# Autodesk Inventor assembly: 21308 E
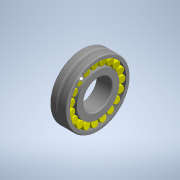
[picture p0: Inventor's stored thumbnail of the model, 180x180]
Saved by Autodesk Inventor 2021 (Build 250183000, 183)
## iProperties
Category: PARTsolutions
Company: SKF
Part Number: 21308 E
Catalog Web Link: www.cadenas.de
Description: BS2_001-Spherical roller bearings
Vendor: SKF
Document SubType Name: Assembly
Designer: partserver
Manufacturer: SKF
Mass: 740 g
Surface Area: 404.704 cm^2
Volume: 89.5824 cm^3
Density: 8.26055 g/cm^3
PSOL_IDENT_0: {$CADENAS_DATA\23d-libs\skf\bearings_units_and_housings\roller_bearings\spherical_roller_bearings\bs
PSOL_IDENT_1: 2_001.prj},173 {VTYP=3D},{STYP=ASSTAB},{NB=21308 E},{LINA=21308 E},{NN=BS2_001},{DATE=23.12.2020 07:
PSOL_IDENT_2: 01:43},{GEOMDATE=14.12.2020 11:44:40},{VERSION=},{LINEID=461840},{WBVAR=},{WBNUMERIC=}  {NB=21308 E}
PSOL_IDENT_3: ,{LINA=21308 E},{KT=DUMMY},{DESIGNATION=21308 E},{VARIANT=CE1W33},{DESIGNX=Cylindrical bore},{SEAL=N
PSOL_IDENT_4: o seals},{SALG=NO},{BORE=40.000},{DD=40.000},{DD1=MIN},{D=90.000},{B=23.000},{DD2=60.000},{DD3=MIN},
PSOL_IDENT_5: {D1=79.800},{B1=MIN},{B2=MIN},{B4=MIN},{B5=MIN},{BB=5.500},{K=3.000},{R12=1.500},{G=},{G1=MIN},{TB=M
PSOL_IDENT_6: IN},{ALPHA=9.0833},{R34=MIN},{PITCH=71.097},{DW=10.200},{LW=8.400},{DDAMIN=49.000},{DDAMAX=MIN},{DBM
PSOL_IDENT_7: IN=MIN},{DAMAX=81.000},{BAMIN=MIN},{RAMAX=1.500},{LOAD1=107.000},{LOAD2=108.000},{LOAD3=11.800},{SPE
PSOL_IDENT_8: ED1=7000},{SPEED2=9500},{PRA=},{PLA=},{Z=19.000},{II=2.000},{MASS=0.740},{MASS2=MIN},{SLEEVE=},{POPU
PSOL_IDENT_9: LAR=Yes},{BEARING=21308 E},{PPATH=parts/bs2_001_asmtpl.prj},{RAMAXX=1.5},{EE=0.24},{Y0=2.8},{R12X=1.
PSOL_IDENT_10: 5},{Y2=4.2},{ALPHAX=9.08333},{Y1=2.8},{DD1X=},{B1X=},{SLEEVEX=},{ALPHAXX=},{B2X=},{SUPRESSED=},{BBAL
PSOL_IDENT_11: G=5.500},{KALG=3.000}
NB: 21308 E
NN: BS2_001
NT: Spherical roller bearings
NBSYN: $DESIGNATION.
LINA: 21308 E
CATALOG: SKF
DESIGNATION: 21308 E
DESIGNX: Cylindrical bore
SEAL: No seals
BORE: 40
D: 90
B: 23
LOAD1: 107
LOAD2: 108
LOAD3: 11.8
SPEED1: 7000
SPEED2: 9500
SUPPLIER: SKF
ARTICLENO: 21308 E
BOMINFO: 21308 E
CREATOR: CADENAS GmbH
Title: 21308 E
Author: Cadenas PARTsolutions
Comments: Spherical roller bearings
## Documents named in this file (6)
- C:\Users\Διογενης Τσιχλακης\Documents\Inventor\GearBoxTurboProp\21308 E.iam
- C:\Users\Διογενης Τσιχλακης\Documents\Inventor\GearBoxTurboProp\21308 E_dummy.ipt
- C:\Users\Διογενης Τσιχλακης\Documents\Inventor\GearBoxTurboProp\21308 E_ir.ipt
- C:\Users\Διογενης Τσιχλακης\Documents\Inventor\GearBoxTurboProp\21308 E_or.ipt
- C:\Users\Διογενης Τσιχλακης\Documents\Inventor\GearBoxTurboProp\21308 E_r1.ipt
- C:\Users\Διογενης Τσιχλακης\Documents\Inventor\GearBoxTurboProp\21308 E_r2.ipt
## Components (41 placed, 5 different names)
1. 21308 E_dummy:1 — dummy_XY@1 <-> ir_XY@2, dummy_Z@1 <-> ir_Z@2, dummy_YZ@1 <-> ir_YZ@2, dummy_YZ@1 <-> or_YZ@3, roller1_XY@1 <-> roller1_XY@4, roller1_Z@1 <-> roller1_Z@4, roller1_YZ@1 <-> roller1_YZ@4, roller1_XY@1 <-> roller2_XY@5, roller1_Z@1 <-> roller2_Z@5, roller1_YZ@1 <-> roller2_YZ@5, roller2_XY@1 <-> roller1_XY@6, roller2_Z@1 <-> roller1_Z@6, roller2_YZ@1 <-> roller1_YZ@6, roller2_XY@1 <-> roller2_XY@7, roller2_Z@1 <-> roller2_Z@7, roller2_YZ@1 <-> roller2_YZ@7, roller3_XY@1 <-> roller1_XY@8, roller3_Z@1 <-> roller1_Z@8, roller3_YZ@1 <-> roller1_YZ@8, roller3_XY@1 <-> roller2_XY@9, roller3_Z@1 <-> roller2_Z@9, roller3_YZ@1 <-> roller2_YZ@9, roller4_XY@1 <-> roller1_XY@10, roller4_Z@1 <-> roller1_Z@10, roller4_YZ@1 <-> roller1_YZ@10, roller4_XY@1 <-> roller2_XY@11, roller4_Z@1 <-> roller2_Z@11, roller4_YZ@1 <-> roller2_YZ@11, roller5_XY@1 <-> roller1_XY@12, roller5_Z@1 <-> roller1_Z@12, roller5_YZ@1 <-> roller1_YZ@12, roller5_XY@1 <-> roller2_XY@13, roller5_Z@1 <-> roller2_Z@13, roller5_YZ@1 <-> roller2_YZ@13, roller6_XY@1 <-> roller1_XY@14, roller6_Z@1 <-> roller1_Z@14, roller6_YZ@1 <-> roller1_YZ@14, roller6_XY@1 <-> roller2_XY@15, roller6_Z@1 <-> roller2_Z@15, roller6_YZ@1 <-> roller2_YZ@15, roller7_XY@1 <-> roller1_XY@16, roller7_Z@1 <-> roller1_Z@16, roller7_YZ@1 <-> roller1_YZ@16, roller7_XY@1 <-> roller2_XY@17, roller7_Z@1 <-> roller2_Z@17, roller7_YZ@1 <-> roller2_YZ@17, roller8_XY@1 <-> roller1_XY@18, roller8_Z@1 <-> roller1_Z@18, roller8_YZ@1 <-> roller1_YZ@18, roller8_XY@1 <-> roller2_XY@19, roller8_Z@1 <-> roller2_Z@19, roller8_YZ@1 <-> roller2_YZ@19, roller9_XY@1 <-> roller1_XY@20, roller9_Z@1 <-> roller1_Z@20, roller9_YZ@1 <-> roller1_YZ@20, roller9_XY@1 <-> roller2_XY@21, roller9_Z@1 <-> roller2_Z@21, roller9_YZ@1 <-> roller2_YZ@21, roller10_XY@1 <-> roller1_XY@22, roller10_Z@1 <-> roller1_Z@22, roller10_YZ@1 <-> roller1_YZ@22, roller10_XY@1 <-> roller2_XY@23, roller10_Z@1 <-> roller2_Z@23, roller10_YZ@1 <-> roller2_YZ@23, roller11_XY@1 <-> roller1_XY@24, roller11_Z@1 <-> roller1_Z@24, roller11_YZ@1 <-> roller1_YZ@24, roller11_XY@1 <-> roller2_XY@25, roller11_Z@1 <-> roller2_Z@25, roller11_YZ@1 <-> roller2_YZ@25, roller12_XY@1 <-> roller1_XY@26, roller12_Z@1 <-> roller1_Z@26, roller12_YZ@1 <-> roller1_YZ@26, roller12_XY@1 <-> roller2_XY@27, roller12_Z@1 <-> roller2_Z@27, roller12_YZ@1 <-> roller2_YZ@27, roller13_XY@1 <-> roller1_XY@28, roller13_Z@1 <-> roller1_Z@28, roller13_YZ@1 <-> roller1_YZ@28, roller13_XY@1 <-> roller2_XY@29, roller13_Z@1 <-> roller2_Z@29, roller13_YZ@1 <-> roller2_YZ@29, roller14_XY@1 <-> roller1_XY@30, roller14_Z@1 <-> roller1_Z@30, roller14_YZ@1 <-> roller1_YZ@30, roller14_XY@1 <-> roller2_XY@31, roller14_Z@1 <-> roller2_Z@31, roller14_YZ@1 <-> roller2_YZ@31, roller15_XY@1 <-> roller1_XY@32, roller15_Z@1 <-> roller1_Z@32, roller15_YZ@1 <-> roller1_YZ@32, roller15_XY@1 <-> roller2_XY@33, roller15_Z@1 <-> roller2_Z@33, roller15_YZ@1 <-> roller2_YZ@33, roller16_XY@1 <-> roller1_XY@34, roller16_Z@1 <-> roller1_Z@34, roller16_YZ@1 <-> roller1_YZ@34, roller16_XY@1 <-> roller2_XY@35, roller16_Z@1 <-> roller2_Z@35, roller16_YZ@1 <-> roller2_YZ@35, roller17_XY@1 <-> roller1_XY@36, roller17_Z@1 <-> roller1_Z@36, roller17_YZ@1 <-> roller1_YZ@36, roller17_XY@1 <-> roller2_XY@37, roller17_Z@1 <-> roller2_Z@37, roller17_YZ@1 <-> roller2_YZ@37, roller18_XY@1 <-> roller1_XY@38, roller18_Z@1 <-> roller1_Z@38, roller18_YZ@1 <-> roller1_YZ@38, roller18_XY@1 <-> roller2_XY@39, roller18_Z@1 <-> roller2_Z@39, roller18_YZ@1 <-> roller2_YZ@39, roller19_XY@1 <-> roller1_XY@40, roller19_Z@1 <-> roller1_Z@40, roller19_YZ@1 <-> roller1_YZ@40, roller19_XY@1 <-> roller2_XY@41, roller19_Z@1 <-> roller2_Z@41, roller19_YZ@1 <-> roller2_YZ@41
2. 21308 E_ir:1 — dummy_XY@1 <-> ir_XY@2, dummy_Z@1 <-> ir_Z@2, dummy_YZ@1 <-> ir_YZ@2, Mate:43, Rotational:1
3. 21308 E_or:1 — dummy_YZ@1 <-> or_YZ@3, Mate:43, Rotational:1
4. 21308 E_r1:1 — roller1_XY@1 <-> roller1_XY@4, roller1_Z@1 <-> roller1_Z@4, roller1_YZ@1 <-> roller1_YZ@4
5. 21308 E_r2:1 — roller1_XY@1 <-> roller2_XY@5, roller1_Z@1 <-> roller2_Z@5, roller1_YZ@1 <-> roller2_YZ@5
6. 21308 E_r1:2 — roller2_XY@1 <-> roller1_XY@6, roller2_Z@1 <-> roller1_Z@6, roller2_YZ@1 <-> roller1_YZ@6
7. 21308 E_r2:2 — roller2_XY@1 <-> roller2_XY@7, roller2_Z@1 <-> roller2_Z@7, roller2_YZ@1 <-> roller2_YZ@7
8. 21308 E_r1:3 — roller3_XY@1 <-> roller1_XY@8, roller3_Z@1 <-> roller1_Z@8, roller3_YZ@1 <-> roller1_YZ@8
9. 21308 E_r2:3 — roller3_XY@1 <-> roller2_XY@9, roller3_Z@1 <-> roller2_Z@9, roller3_YZ@1 <-> roller2_YZ@9
10. 21308 E_r1:4 — roller4_XY@1 <-> roller1_XY@10, roller4_Z@1 <-> roller1_Z@10, roller4_YZ@1 <-> roller1_YZ@10
11. 21308 E_r2:4 — roller4_XY@1 <-> roller2_XY@11, roller4_Z@1 <-> roller2_Z@11, roller4_YZ@1 <-> roller2_YZ@11
12. 21308 E_r1:5 — roller5_XY@1 <-> roller1_XY@12, roller5_Z@1 <-> roller1_Z@12, roller5_YZ@1 <-> roller1_YZ@12
13. 21308 E_r2:5 — roller5_XY@1 <-> roller2_XY@13, roller5_Z@1 <-> roller2_Z@13, roller5_YZ@1 <-> roller2_YZ@13
14. 21308 E_r1:6 — roller6_XY@1 <-> roller1_XY@14, roller6_Z@1 <-> roller1_Z@14, roller6_YZ@1 <-> roller1_YZ@14
15. 21308 E_r2:6 — roller6_XY@1 <-> roller2_XY@15, roller6_Z@1 <-> roller2_Z@15, roller6_YZ@1 <-> roller2_YZ@15
16. 21308 E_r1:7 — roller7_XY@1 <-> roller1_XY@16, roller7_Z@1 <-> roller1_Z@16, roller7_YZ@1 <-> roller1_YZ@16
17. 21308 E_r2:7 — roller7_XY@1 <-> roller2_XY@17, roller7_Z@1 <-> roller2_Z@17, roller7_YZ@1 <-> roller2_YZ@17
18. 21308 E_r1:8 — roller8_XY@1 <-> roller1_XY@18, roller8_Z@1 <-> roller1_Z@18, roller8_YZ@1 <-> roller1_YZ@18
19. 21308 E_r2:8 — roller8_XY@1 <-> roller2_XY@19, roller8_Z@1 <-> roller2_Z@19, roller8_YZ@1 <-> roller2_YZ@19
20. 21308 E_r1:9 — roller9_XY@1 <-> roller1_XY@20, roller9_Z@1 <-> roller1_Z@20, roller9_YZ@1 <-> roller1_YZ@20
21. 21308 E_r2:9 — roller9_XY@1 <-> roller2_XY@21, roller9_Z@1 <-> roller2_Z@21, roller9_YZ@1 <-> roller2_YZ@21
22. 21308 E_r1:10 — roller10_XY@1 <-> roller1_XY@22, roller10_Z@1 <-> roller1_Z@22, roller10_YZ@1 <-> roller1_YZ@22
23. 21308 E_r2:10 — roller10_XY@1 <-> roller2_XY@23, roller10_Z@1 <-> roller2_Z@23, roller10_YZ@1 <-> roller2_YZ@23
24. 21308 E_r1:11 — roller11_XY@1 <-> roller1_XY@24, roller11_Z@1 <-> roller1_Z@24, roller11_YZ@1 <-> roller1_YZ@24
25. 21308 E_r2:11 — roller11_XY@1 <-> roller2_XY@25, roller11_Z@1 <-> roller2_Z@25, roller11_YZ@1 <-> roller2_YZ@25
26. 21308 E_r1:12 — roller12_XY@1 <-> roller1_XY@26, roller12_Z@1 <-> roller1_Z@26, roller12_YZ@1 <-> roller1_YZ@26
27. 21308 E_r2:12 — roller12_XY@1 <-> roller2_XY@27, roller12_Z@1 <-> roller2_Z@27, roller12_YZ@1 <-> roller2_YZ@27
28. 21308 E_r1:13 — roller13_XY@1 <-> roller1_XY@28, roller13_Z@1 <-> roller1_Z@28, roller13_YZ@1 <-> roller1_YZ@28
29. 21308 E_r2:13 — roller13_XY@1 <-> roller2_XY@29, roller13_Z@1 <-> roller2_Z@29, roller13_YZ@1 <-> roller2_YZ@29
30. 21308 E_r1:14 — roller14_XY@1 <-> roller1_XY@30, roller14_Z@1 <-> roller1_Z@30, roller14_YZ@1 <-> roller1_YZ@30
31. 21308 E_r2:14 — roller14_XY@1 <-> roller2_XY@31, roller14_Z@1 <-> roller2_Z@31, roller14_YZ@1 <-> roller2_YZ@31
32. 21308 E_r1:15 — roller15_XY@1 <-> roller1_XY@32, roller15_Z@1 <-> roller1_Z@32, roller15_YZ@1 <-> roller1_YZ@32
33. 21308 E_r2:15 — roller15_XY@1 <-> roller2_XY@33, roller15_Z@1 <-> roller2_Z@33, roller15_YZ@1 <-> roller2_YZ@33
34. 21308 E_r1:16 — roller16_XY@1 <-> roller1_XY@34, roller16_Z@1 <-> roller1_Z@34, roller16_YZ@1 <-> roller1_YZ@34
35. 21308 E_r2:16 — roller16_XY@1 <-> roller2_XY@35, roller16_Z@1 <-> roller2_Z@35, roller16_YZ@1 <-> roller2_YZ@35
36. 21308 E_r1:17 — roller17_XY@1 <-> roller1_XY@36, roller17_Z@1 <-> roller1_Z@36, roller17_YZ@1 <-> roller1_YZ@36
37. 21308 E_r2:17 — roller17_XY@1 <-> roller2_XY@37, roller17_Z@1 <-> roller2_Z@37, roller17_YZ@1 <-> roller2_YZ@37
38. 21308 E_r1:18 — roller18_XY@1 <-> roller1_XY@38, roller18_Z@1 <-> roller1_Z@38, roller18_YZ@1 <-> roller1_YZ@38
39. 21308 E_r2:18 — roller18_XY@1 <-> roller2_XY@39, roller18_Z@1 <-> roller2_Z@39, roller18_YZ@1 <-> roller2_YZ@39
40. 21308 E_r1:19 — roller19_XY@1 <-> roller1_XY@40, roller19_Z@1 <-> roller1_Z@40, roller19_YZ@1 <-> roller1_YZ@40
41. 21308 E_r2:19 — roller19_XY@1 <-> roller2_XY@41, roller19_Z@1 <-> roller2_Z@41, roller19_YZ@1 <-> roller2_YZ@41
## Relationships (120: Mate 41, Angle 40, Flush 38, RevoluteJoint 1)
- dummy_XY@1 <-> ir_XY@2 [Mate]: 21308 E_dummy:1 ↔ 21308 E_ir:1
- dummy_Z@1 <-> ir_Z@2 [Mate]: 21308 E_dummy:1 ↔ 21308 E_ir:1
- dummy_YZ@1 <-> ir_YZ@2 [Angle] (0 deg): 21308 E_dummy:1 ↔ 21308 E_ir:1
- dummy_YZ@1 <-> or_YZ@3 [Angle] (0 deg): 21308 E_dummy:1 ↔ 21308 E_or:1
- roller1_XY@1 <-> roller1_XY@4 [Flush]: 21308 E_dummy:1 ↔ 21308 E_r1:1
- roller1_Z@1 <-> roller1_Z@4 [Mate]: 21308 E_dummy:1 ↔ 21308 E_r1:1
- roller1_YZ@1 <-> roller1_YZ@4 [Angle] (0 deg): 21308 E_dummy:1 ↔ 21308 E_r1:1
- roller1_XY@1 <-> roller2_XY@5 [Flush]: 21308 E_dummy:1 ↔ 21308 E_r2:1
- roller1_Z@1 <-> roller2_Z@5 [Mate]: 21308 E_dummy:1 ↔ 21308 E_r2:1
- roller1_YZ@1 <-> roller2_YZ@5 [Angle] (0 deg): 21308 E_dummy:1 ↔ 21308 E_r2:1
- roller2_XY@1 <-> roller1_XY@6 [Flush]: 21308 E_dummy:1 ↔ 21308 E_r1:2
- roller2_Z@1 <-> roller1_Z@6 [Mate]: 21308 E_dummy:1 ↔ 21308 E_r1:2
- roller2_YZ@1 <-> roller1_YZ@6 [Angle] (0 deg): 21308 E_dummy:1 ↔ 21308 E_r1:2
- roller2_XY@1 <-> roller2_XY@7 [Flush]: 21308 E_dummy:1 ↔ 21308 E_r2:2
- roller2_Z@1 <-> roller2_Z@7 [Mate]: 21308 E_dummy:1 ↔ 21308 E_r2:2
- roller2_YZ@1 <-> roller2_YZ@7 [Angle] (0 deg): 21308 E_dummy:1 ↔ 21308 E_r2:2
- roller3_XY@1 <-> roller1_XY@8 [Flush]: 21308 E_dummy:1 ↔ 21308 E_r1:3
- roller3_Z@1 <-> roller1_Z@8 [Mate]: 21308 E_dummy:1 ↔ 21308 E_r1:3
- roller3_YZ@1 <-> roller1_YZ@8 [Angle] (0 deg): 21308 E_dummy:1 ↔ 21308 E_r1:3
- roller3_XY@1 <-> roller2_XY@9 [Flush]: 21308 E_dummy:1 ↔ 21308 E_r2:3
- roller3_Z@1 <-> roller2_Z@9 [Mate]: 21308 E_dummy:1 ↔ 21308 E_r2:3
- roller3_YZ@1 <-> roller2_YZ@9 [Angle] (0 deg): 21308 E_dummy:1 ↔ 21308 E_r2:3
- roller4_XY@1 <-> roller1_XY@10 [Flush]: 21308 E_dummy:1 ↔ 21308 E_r1:4
- roller4_Z@1 <-> roller1_Z@10 [Mate]: 21308 E_dummy:1 ↔ 21308 E_r1:4
- roller4_YZ@1 <-> roller1_YZ@10 [Angle] (0 deg): 21308 E_dummy:1 ↔ 21308 E_r1:4
- roller4_XY@1 <-> roller2_XY@11 [Flush]: 21308 E_dummy:1 ↔ 21308 E_r2:4
- roller4_Z@1 <-> roller2_Z@11 [Mate]: 21308 E_dummy:1 ↔ 21308 E_r2:4
- roller4_YZ@1 <-> roller2_YZ@11 [Angle] (0 deg): 21308 E_dummy:1 ↔ 21308 E_r2:4
- roller5_XY@1 <-> roller1_XY@12 [Flush]: 21308 E_dummy:1 ↔ 21308 E_r1:5
- roller5_Z@1 <-> roller1_Z@12 [Mate]: 21308 E_dummy:1 ↔ 21308 E_r1:5
- roller5_YZ@1 <-> roller1_YZ@12 [Angle] (0 deg): 21308 E_dummy:1 ↔ 21308 E_r1:5
- roller5_XY@1 <-> roller2_XY@13 [Flush]: 21308 E_dummy:1 ↔ 21308 E_r2:5
- roller5_Z@1 <-> roller2_Z@13 [Mate]: 21308 E_dummy:1 ↔ 21308 E_r2:5
- roller5_YZ@1 <-> roller2_YZ@13 [Angle] (0 deg): 21308 E_dummy:1 ↔ 21308 E_r2:5
- roller6_XY@1 <-> roller1_XY@14 [Flush]: 21308 E_dummy:1 ↔ 21308 E_r1:6
- roller6_Z@1 <-> roller1_Z@14 [Mate]: 21308 E_dummy:1 ↔ 21308 E_r1:6
- roller6_YZ@1 <-> roller1_YZ@14 [Angle] (0 deg): 21308 E_dummy:1 ↔ 21308 E_r1:6
- roller6_XY@1 <-> roller2_XY@15 [Flush]: 21308 E_dummy:1 ↔ 21308 E_r2:6
- roller6_Z@1 <-> roller2_Z@15 [Mate]: 21308 E_dummy:1 ↔ 21308 E_r2:6
- roller6_YZ@1 <-> roller2_YZ@15 [Angle] (0 deg): 21308 E_dummy:1 ↔ 21308 E_r2:6
- roller7_XY@1 <-> roller1_XY@16 [Flush]: 21308 E_dummy:1 ↔ 21308 E_r1:7
- roller7_Z@1 <-> roller1_Z@16 [Mate]: 21308 E_dummy:1 ↔ 21308 E_r1:7
- roller7_YZ@1 <-> roller1_YZ@16 [Angle] (0 deg): 21308 E_dummy:1 ↔ 21308 E_r1:7
- roller7_XY@1 <-> roller2_XY@17 [Flush]: 21308 E_dummy:1 ↔ 21308 E_r2:7
- roller7_Z@1 <-> roller2_Z@17 [Mate]: 21308 E_dummy:1 ↔ 21308 E_r2:7
- roller7_YZ@1 <-> roller2_YZ@17 [Angle] (0 deg): 21308 E_dummy:1 ↔ 21308 E_r2:7
- roller8_XY@1 <-> roller1_XY@18 [Flush]: 21308 E_dummy:1 ↔ 21308 E_r1:8
- roller8_Z@1 <-> roller1_Z@18 [Mate]: 21308 E_dummy:1 ↔ 21308 E_r1:8
- roller8_YZ@1 <-> roller1_YZ@18 [Angle] (0 deg): 21308 E_dummy:1 ↔ 21308 E_r1:8
- roller8_XY@1 <-> roller2_XY@19 [Flush]: 21308 E_dummy:1 ↔ 21308 E_r2:8
- roller8_Z@1 <-> roller2_Z@19 [Mate]: 21308 E_dummy:1 ↔ 21308 E_r2:8
- roller8_YZ@1 <-> roller2_YZ@19 [Angle] (0 deg): 21308 E_dummy:1 ↔ 21308 E_r2:8
- roller9_XY@1 <-> roller1_XY@20 [Flush]: 21308 E_dummy:1 ↔ 21308 E_r1:9
- roller9_Z@1 <-> roller1_Z@20 [Mate]: 21308 E_dummy:1 ↔ 21308 E_r1:9
- roller9_YZ@1 <-> roller1_YZ@20 [Angle] (0 deg): 21308 E_dummy:1 ↔ 21308 E_r1:9
- roller9_XY@1 <-> roller2_XY@21 [Flush]: 21308 E_dummy:1 ↔ 21308 E_r2:9
- roller9_Z@1 <-> roller2_Z@21 [Mate]: 21308 E_dummy:1 ↔ 21308 E_r2:9
- roller9_YZ@1 <-> roller2_YZ@21 [Angle] (0 deg): 21308 E_dummy:1 ↔ 21308 E_r2:9
- roller10_XY@1 <-> roller1_XY@22 [Flush]: 21308 E_dummy:1 ↔ 21308 E_r1:10
- roller10_Z@1 <-> roller1_Z@22 [Mate]: 21308 E_dummy:1 ↔ 21308 E_r1:10
- roller10_YZ@1 <-> roller1_YZ@22 [Angle] (0 deg): 21308 E_dummy:1 ↔ 21308 E_r1:10
- roller10_XY@1 <-> roller2_XY@23 [Flush]: 21308 E_dummy:1 ↔ 21308 E_r2:10
- roller10_Z@1 <-> roller2_Z@23 [Mate]: 21308 E_dummy:1 ↔ 21308 E_r2:10
- roller10_YZ@1 <-> roller2_YZ@23 [Angle] (0 deg): 21308 E_dummy:1 ↔ 21308 E_r2:10
- roller11_XY@1 <-> roller1_XY@24 [Flush]: 21308 E_dummy:1 ↔ 21308 E_r1:11
- roller11_Z@1 <-> roller1_Z@24 [Mate]: 21308 E_dummy:1 ↔ 21308 E_r1:11
- roller11_YZ@1 <-> roller1_YZ@24 [Angle] (0 deg): 21308 E_dummy:1 ↔ 21308 E_r1:11
- roller11_XY@1 <-> roller2_XY@25 [Flush]: 21308 E_dummy:1 ↔ 21308 E_r2:11
- roller11_Z@1 <-> roller2_Z@25 [Mate]: 21308 E_dummy:1 ↔ 21308 E_r2:11
- roller11_YZ@1 <-> roller2_YZ@25 [Angle] (0 deg): 21308 E_dummy:1 ↔ 21308 E_r2:11
- roller12_XY@1 <-> roller1_XY@26 [Flush]: 21308 E_dummy:1 ↔ 21308 E_r1:12
- roller12_Z@1 <-> roller1_Z@26 [Mate]: 21308 E_dummy:1 ↔ 21308 E_r1:12
- roller12_YZ@1 <-> roller1_YZ@26 [Angle] (0 deg): 21308 E_dummy:1 ↔ 21308 E_r1:12
- roller12_XY@1 <-> roller2_XY@27 [Flush]: 21308 E_dummy:1 ↔ 21308 E_r2:12
- roller12_Z@1 <-> roller2_Z@27 [Mate]: 21308 E_dummy:1 ↔ 21308 E_r2:12
- roller12_YZ@1 <-> roller2_YZ@27 [Angle] (0 deg): 21308 E_dummy:1 ↔ 21308 E_r2:12
- roller13_XY@1 <-> roller1_XY@28 [Flush]: 21308 E_dummy:1 ↔ 21308 E_r1:13
- roller13_Z@1 <-> roller1_Z@28 [Mate]: 21308 E_dummy:1 ↔ 21308 E_r1:13
- roller13_YZ@1 <-> roller1_YZ@28 [Angle] (0 deg): 21308 E_dummy:1 ↔ 21308 E_r1:13
- roller13_XY@1 <-> roller2_XY@29 [Flush]: 21308 E_dummy:1 ↔ 21308 E_r2:13
- roller13_Z@1 <-> roller2_Z@29 [Mate]: 21308 E_dummy:1 ↔ 21308 E_r2:13
- roller13_YZ@1 <-> roller2_YZ@29 [Angle] (0 deg): 21308 E_dummy:1 ↔ 21308 E_r2:13
- roller14_XY@1 <-> roller1_XY@30 [Flush]: 21308 E_dummy:1 ↔ 21308 E_r1:14
- roller14_Z@1 <-> roller1_Z@30 [Mate]: 21308 E_dummy:1 ↔ 21308 E_r1:14
- roller14_YZ@1 <-> roller1_YZ@30 [Angle] (0 deg): 21308 E_dummy:1 ↔ 21308 E_r1:14
- roller14_XY@1 <-> roller2_XY@31 [Flush]: 21308 E_dummy:1 ↔ 21308 E_r2:14
- roller14_Z@1 <-> roller2_Z@31 [Mate]: 21308 E_dummy:1 ↔ 21308 E_r2:14
- roller14_YZ@1 <-> roller2_YZ@31 [Angle] (0 deg): 21308 E_dummy:1 ↔ 21308 E_r2:14
- roller15_XY@1 <-> roller1_XY@32 [Flush]: 21308 E_dummy:1 ↔ 21308 E_r1:15
- roller15_Z@1 <-> roller1_Z@32 [Mate]: 21308 E_dummy:1 ↔ 21308 E_r1:15
- roller15_YZ@1 <-> roller1_YZ@32 [Angle] (0 deg): 21308 E_dummy:1 ↔ 21308 E_r1:15
- roller15_XY@1 <-> roller2_XY@33 [Flush]: 21308 E_dummy:1 ↔ 21308 E_r2:15
- roller15_Z@1 <-> roller2_Z@33 [Mate]: 21308 E_dummy:1 ↔ 21308 E_r2:15
- roller15_YZ@1 <-> roller2_YZ@33 [Angle] (0 deg): 21308 E_dummy:1 ↔ 21308 E_r2:15
- roller16_XY@1 <-> roller1_XY@34 [Flush]: 21308 E_dummy:1 ↔ 21308 E_r1:16
- roller16_Z@1 <-> roller1_Z@34 [Mate]: 21308 E_dummy:1 ↔ 21308 E_r1:16
- roller16_YZ@1 <-> roller1_YZ@34 [Angle] (0 deg): 21308 E_dummy:1 ↔ 21308 E_r1:16
- roller16_XY@1 <-> roller2_XY@35 [Flush]: 21308 E_dummy:1 ↔ 21308 E_r2:16
- roller16_Z@1 <-> roller2_Z@35 [Mate]: 21308 E_dummy:1 ↔ 21308 E_r2:16
- roller16_YZ@1 <-> roller2_YZ@35 [Angle] (0 deg): 21308 E_dummy:1 ↔ 21308 E_r2:16
- roller17_XY@1 <-> roller1_XY@36 [Flush]: 21308 E_dummy:1 ↔ 21308 E_r1:17
- roller17_Z@1 <-> roller1_Z@36 [Mate]: 21308 E_dummy:1 ↔ 21308 E_r1:17
- roller17_YZ@1 <-> roller1_YZ@36 [Angle] (0 deg): 21308 E_dummy:1 ↔ 21308 E_r1:17
- roller17_XY@1 <-> roller2_XY@37 [Flush]: 21308 E_dummy:1 ↔ 21308 E_r2:17
- roller17_Z@1 <-> roller2_Z@37 [Mate]: 21308 E_dummy:1 ↔ 21308 E_r2:17
- roller17_YZ@1 <-> roller2_YZ@37 [Angle] (0 deg): 21308 E_dummy:1 ↔ 21308 E_r2:17
- roller18_XY@1 <-> roller1_XY@38 [Flush]: 21308 E_dummy:1 ↔ 21308 E_r1:18
- roller18_Z@1 <-> roller1_Z@38 [Mate]: 21308 E_dummy:1 ↔ 21308 E_r1:18
- roller18_YZ@1 <-> roller1_YZ@38 [Angle] (0 deg): 21308 E_dummy:1 ↔ 21308 E_r1:18
- roller18_XY@1 <-> roller2_XY@39 [Flush]: 21308 E_dummy:1 ↔ 21308 E_r2:18
- roller18_Z@1 <-> roller2_Z@39 [Mate]: 21308 E_dummy:1 ↔ 21308 E_r2:18
- roller18_YZ@1 <-> roller2_YZ@39 [Angle] (0 deg): 21308 E_dummy:1 ↔ 21308 E_r2:18
- roller19_XY@1 <-> roller1_XY@40 [Flush]: 21308 E_dummy:1 ↔ 21308 E_r1:19
- roller19_Z@1 <-> roller1_Z@40 [Mate]: 21308 E_dummy:1 ↔ 21308 E_r1:19
- roller19_YZ@1 <-> roller1_YZ@40 [Angle] (0 deg): 21308 E_dummy:1 ↔ 21308 E_r1:19
- roller19_XY@1 <-> roller2_XY@41 [Flush]: 21308 E_dummy:1 ↔ 21308 E_r2:19
- roller19_Z@1 <-> roller2_Z@41 [Mate]: 21308 E_dummy:1 ↔ 21308 E_r2:19
- roller19_YZ@1 <-> roller2_YZ@41 [Angle] (0 deg): 21308 E_dummy:1 ↔ 21308 E_r2:19
- Mate:43: 21308 E_ir:1 ↔ 21308 E_or:1
- Rotational:1 [RevoluteJoint]: 21308 E_ir:1 ↔ 21308 E_or:1
